# Autodesk Inventor assembly: Zespół14
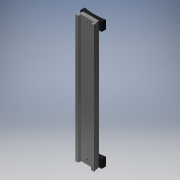
[picture p0: Inventor's stored thumbnail of the model, 180x180]
Saved by Autodesk Inventor 2019.4 (Build 234330000, 330)
## iProperties
Created: 2019-06-02
Part Number: Zespół14
Material: Ogólny
Document SubType Name: Assembly
Designer: barto
Author: barto
## Documents named in this file (3)
- F:\GOTOWY BEM\Złożenie tuba\Zespół14.iam
- F:\GOTOWY BEM\Złożenie tuba\szyna.ipt
- F:\GOTOWY BEM\Złożenie tuba\podkladka.ipt
## Components (3 placed, 2 different names)
1. szyna:1 — Zestawiające:1, Zestawiające:2, Zestawiające:3, Zestawiające:4
2. podkladka:1 — Zestawiające:2, Zestawiające:3
3. podkladka:2 — Zestawiające:1, Zestawiające:4
## Relationships (4: Mate 4)
- Zestawiające:1 [Mate]: szyna:1 ↔ podkladka:2
- Zestawiające:2 [Mate]: szyna:1 ↔ podkladka:1
- Zestawiające:3 [Mate]: szyna:1 ↔ podkladka:1
- Zestawiające:4 [Mate]: szyna:1 ↔ podkladka:2
